# Autodesk Inventor assembly: NASA-20-MM
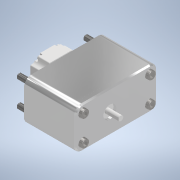
[picture p0: Inventor's stored thumbnail of the model, 180x180]
Saved by Autodesk Inventor 2020 (Build 240168000, 168)
## iProperties
Created: 2019-09-22
Part Number: NASA-20-MM
Document SubType Name: Assembly
Designer: Rick Szalay
Author: Rick Szalay
## Documents named in this file (5)
- C:\Users\Rick Szalay\Documents\NASA-20\NASA-20\MM\NASA-20-MM.iam
- C:\Users\Rick Szalay\Documents\NASA-20\NASA-20\MM\NASA-20-MM-MB-01.ipt
- C:\Users\Rick Szalay\Documents\NASA-20\NASA-20\A428.ipt
- C:\Users\Rick Szalay\Documents\NASA-20\NASA-20\MM\NASA-20-MM-MP-01.ipt
- C:\Users\Rick Szalay\Documents\Inventor\Content Center Files\R2020\en-US\ANSI B18.3(05)\ANSI B18.3 - 1_4-20 UNC - 3(31).ipt
## Components (7 placed, 4 different names)
1. NASA-20-MM-MB-01:1 — Flush:1, Mate:1, Mate:2, Mate:3, Flush:2, Flush:3
2. A428:1 — Flush:1, Mate:1, Mate:2
3. NASA-20-MM-MP-01:1 — Mate:3, Flush:2, Flush:3, Insert:1, Insert:2, Insert:3, Insert:4
4. Hexagon Socket Head Cap Screw - Inch 1/4 - 20 UNC - 3:1 — Insert:1
5. Hexagon Socket Head Cap Screw - Inch 1/4 - 20 UNC - 3:2 — Insert:2
6. Hexagon Socket Head Cap Screw - Inch 1/4 - 20 UNC - 3:3 — Insert:3
7. Hexagon Socket Head Cap Screw - Inch 1/4 - 20 UNC - 3:4 — Insert:4
## Relationships (10: Insert 4, Flush 3, Mate 3)
- Flush:1: NASA-20-MM-MB-01:1 ↔ A428:1
- Mate:1: NASA-20-MM-MB-01:1 ↔ A428:1
- Mate:2: NASA-20-MM-MB-01:1 ↔ A428:1
- Mate:3: NASA-20-MM-MB-01:1 ↔ NASA-20-MM-MP-01:1
- Flush:2: NASA-20-MM-MB-01:1 ↔ NASA-20-MM-MP-01:1
- Flush:3: NASA-20-MM-MB-01:1 ↔ NASA-20-MM-MP-01:1
- Insert:1: NASA-20-MM-MP-01:1 ↔ Hexagon Socket Head Cap Screw - Inch 1/4 - 20 UNC - 3:1
- Insert:2: NASA-20-MM-MP-01:1 ↔ Hexagon Socket Head Cap Screw - Inch 1/4 - 20 UNC - 3:2
- Insert:3: NASA-20-MM-MP-01:1 ↔ Hexagon Socket Head Cap Screw - Inch 1/4 - 20 UNC - 3:3
- Insert:4: NASA-20-MM-MP-01:1 ↔ Hexagon Socket Head Cap Screw - Inch 1/4 - 20 UNC - 3:4
